# Autodesk Inventor assembly: Assembly1
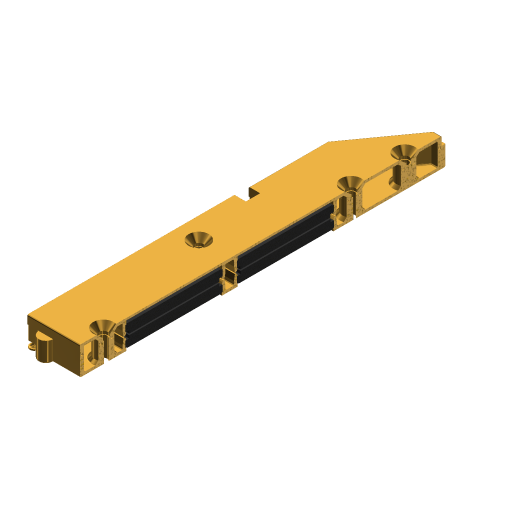
[picture p0: Inventor's stored thumbnail of the model, 512x512]
Saved by Autodesk Inventor 2024.3 (Build 283343000, 343)
## iProperties
Created: 2024-09-21
Part Number: Assembly1
Document SubType Name: Assembly
Designer: User
Author: User
## Documents named in this file (5)
- C:\Users\User\Desktop\Notebook\Speaker Assembly.iam
- C:\Users\User\Desktop\Notebook\Speaker Housing\Upside.ipt
- C:\Users\User\Desktop\Notebook\Speaker Housing\Downside.ipt
- C:\Users\User\Desktop\Notebook\Speaker Driver.ipt
- C:\Users\User\Desktop\Notebook\Speaker Housing.ipt
## Components (6 placed, 3 different names)
1. Upside:1 — Flush:1, Flush:2, Flush:3, Mate:2, Mate:3, Mate:5, Mate:6, Insert:1, Insert:2, Mate:15, Mate:16
2. Downside:2 — Mate:8, Mate:9, Mate:11, Mate:12, Insert:1, Insert:2, Mate:13, Mate:14
3. Speaker Driver:1 — Mate:2, Mate:3, Mate:15
4. Speaker Driver:2 — Mate:8, Mate:9, Mate:13
5. Speaker Driver:3 — Mate:11, Mate:12, Mate:14
6. Speaker Driver:4 — Mate:5, Mate:6, Mate:16
## Relationships (17: Mate 12, Flush 3, Insert 2)
- Flush:1: Upside:1
- Flush:2: Upside:1
- Flush:3: Upside:1
- Mate:2: Upside:1 ↔ Speaker Driver:1
- Mate:3: Upside:1 ↔ Speaker Driver:1
- Mate:5: Upside:1 ↔ Speaker Driver:4
- Mate:6: Upside:1 ↔ Speaker Driver:4
- Mate:8: Downside:2 ↔ Speaker Driver:2
- Mate:9: Downside:2 ↔ Speaker Driver:2
- Mate:11: Downside:2 ↔ Speaker Driver:3
- Mate:12: Downside:2 ↔ Speaker Driver:3
- Insert:1: Upside:1 ↔ Downside:2
- Insert:2: Upside:1 ↔ Downside:2
- Mate:13: Downside:2 ↔ Speaker Driver:2
- Mate:14: Downside:2 ↔ Speaker Driver:3
- Mate:15: Upside:1 ↔ Speaker Driver:1
- Mate:16: Upside:1 ↔ Speaker Driver:4
